# Autodesk Inventor assembly: Lightsaber Assembly
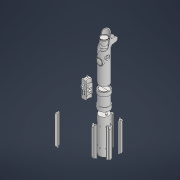
[picture p0: Inventor's stored thumbnail of the model, 180x180]
Saved by Autodesk Inventor 2021 (Build 250183000, 183)
## iProperties
Created: 2021-01-08
Part Number: Lightsaber Assembly
Document SubType Name: Assembly
Designer: Alex
Author: Alex
## Documents named in this file (12)
- C:\Users\Alex\Downloads\Lightsaber Assembly.iam
- C:\Users\Alex\Downloads\Grip Base.ipt
- C:\Users\Alex\Downloads\Grip.ipt
- C:\Users\Alex\Downloads\Middle handle.ipt
- C:\Users\Alex\Downloads\Button.ipt
- C:\Users\Alex\Downloads\Switch.ipt
- C:\Users\Alex\Downloads\top.ipt
- C:\Users\Alex\Downloads\emitter.ipt
- C:\Users\Alex\Downloads\Button1.ipt
- C:\Users\Alex\Downloads\Pin2.ipt
- C:\Users\Alex\Downloads\Clip.ipt
- C:\Users\Alex\Downloads\pin.ipt
## Components (20 placed, 11 different names)
1. Grip Base:1 — Flush:1, Flush:2, Mate:2, Flush:3, Flush:4, Flush:5, Flush:6, Mate:8, Mate:17, Mate:24, Mate:25, Mate:26, Mate:27, Mate:28, Mate:29, Insert:1, Insert:2
2. Grip:1 — Flush:1, Mate:29
3. Grip:2 — Flush:2, Mate:2, Mate:24
4. Grip:3 — Flush:4, Mate:26
5. Grip:4 — Flush:5, Mate:27
6. Grip:5 — Flush:3, Mate:28
7. Grip:6 — Flush:6, Mate:25, Mate:33, Mate:34
8. Middle handle:1 — Mate:8, Mate:9, Flush:7, Mate:13, Mate:16, Mate:17
9. Button:1 — Mate:9, Flush:7, Mate:10, Mate:11, Mate:12
10. Switch:1 — Mate:10, Mate:11, Mate:12
11. top:1 — Mate:13, Mate:14, Mate:15, Mate:16, Mate:18, Mate:19, Mate:20, Mate:21, Mate:22, Mate:23, Mate:30, Mate:31, Mate:32
12. emitter:1 — Mate:14, Mate:15
13. Button1:1 — Mate:18, Mate:19
14. Pin2:1 — Mate:20, Flush:8
15. Pin2:2 — Mate:21, Flush:8
16. Pin2:3 — Mate:22
17. Pin2:4 — Mate:23
18. Clip:1 — Mate:30, Mate:31, Mate:32
19. pin:1 — Insert:1, Mate:33
20. pin:2 — Insert:2, Mate:34
## Relationships (38: Mate 28, Flush 8, Insert 2)
- Flush:1: Grip Base:1 ↔ Grip:1
- Flush:2: Grip Base:1 ↔ Grip:2
- Mate:2: Grip Base:1 ↔ Grip:2
- Flush:3: Grip Base:1 ↔ Grip:5
- Flush:4: Grip Base:1 ↔ Grip:3
- Flush:5: Grip Base:1 ↔ Grip:4
- Flush:6: Grip Base:1 ↔ Grip:6
- Mate:8: Grip Base:1 ↔ Middle handle:1
- Mate:9: Middle handle:1 ↔ Button:1
- Flush:7: Middle handle:1 ↔ Button:1
- Mate:10 (1 mm): Button:1 ↔ Switch:1
- Mate:11 (1 mm): Button:1 ↔ Switch:1
- Mate:12 (1 mm): Button:1 ↔ Switch:1
- Mate:13: Middle handle:1 ↔ top:1
- Mate:14: top:1 ↔ emitter:1
- Mate:15: top:1 ↔ emitter:1
- Mate:16: Middle handle:1 ↔ top:1
- Mate:17: Grip Base:1 ↔ Middle handle:1
- Mate:18: top:1 ↔ Button1:1
- Mate:19: top:1 ↔ Button1:1
- Mate:20: top:1 ↔ Pin2:1
- Mate:21: top:1 ↔ Pin2:2
- Flush:8: Pin2:1 ↔ Pin2:2
- Mate:22: top:1 ↔ Pin2:3
- Mate:23: top:1 ↔ Pin2:4
- Mate:24: Grip Base:1 ↔ Grip:2
- Mate:25: Grip Base:1 ↔ Grip:6
- Mate:26: Grip Base:1 ↔ Grip:3
- Mate:27: Grip Base:1 ↔ Grip:4
- Mate:28: Grip Base:1 ↔ Grip:5
- Mate:29: Grip Base:1 ↔ Grip:1
- Mate:30: top:1 ↔ Clip:1
- Mate:31: top:1 ↔ Clip:1
- Mate:32: top:1 ↔ Clip:1
- Insert:1: Grip Base:1 ↔ pin:1
- Mate:33: Grip:6 ↔ pin:1
- Insert:2: Grip Base:1 ↔ pin:2
- Mate:34 (0.1 mm): Grip:6 ↔ pin:2
